# Autodesk Inventor assembly: Assembly8
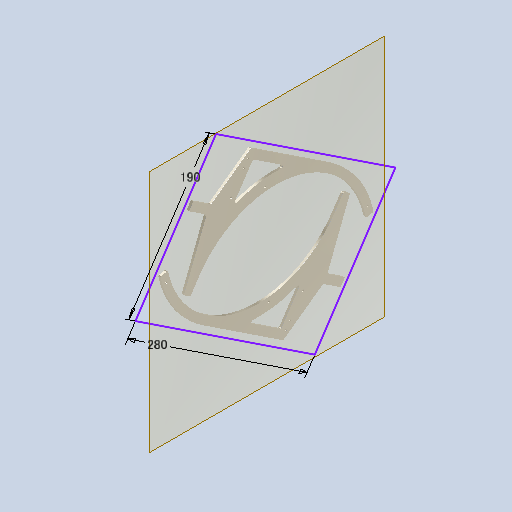
[picture p0: Inventor's stored thumbnail of the model, 512x512]
Saved by Autodesk Inventor 2025.2 (Build 292293000, 293)
## iProperties
Created: 2024-12-26
Part Number: Assembly8
Document SubType Name: Assembly
Designer: haruy
Author: haruy
## Documents named in this file (2)
- C:\Users\haruy\Documents\ロボコン\NHK2025\cad\cnc\Assembly8.iam
- C:\Users\haruy\Documents\ロボコン\NHK2025\cad\nagahisa\belt_liner\belt_liner_v1_Plate_10.ipt
## Components (2 placed, 1 different names)
1. belt_liner_v1_Plate_10:1 — フラッシュ:1
2. belt_liner_v1_Plate_10:2 — フラッシュ:2
## Relationships (2: Flush 2)
- フラッシュ:1 [Flush]: belt_liner_v1_Plate_10:1
- フラッシュ:2 [Flush]: belt_liner_v1_Plate_10:2
